# Autodesk Inventor assembly: Printhead Assembly
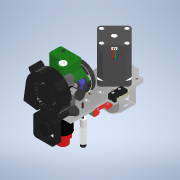
[picture p0: Inventor's stored thumbnail of the model, 180x180]
Saved by Autodesk Inventor 2020 (Build 240168000, 168)
## iProperties
Created: 2023-06-15
Part Number: Printhead Assembly
Document SubType Name: Assembly
Designer: Ishaan
Author: Ishaan
## Documents named in this file (16)
- D:\Documents\Projects\Axiom - IDEX 3D Printer\CAD\01 - Printhead\Printhead Assembly.iam
- D:\Documents\Projects\Axiom - IDEX 3D Printer\CAD\01 - Printhead\Printhead Base Plate REVI.ipt
- D:\Documents\Projects\Axiom - IDEX 3D Printer\CAD\00 - COTS Components\Orbiter Extruder\Orbiter Extruder with Sensor.iam
- D:\Documents\Projects\Axiom - IDEX 3D Printer\CAD\00 - COTS Components\CHC Hotend\TD6S-CHC_mockup.iam
- D:\Documents\Projects\Axiom - IDEX 3D Printer\CAD\00 - COTS Components\3010 Fan\Fan 3010.ipt
- D:\Documents\Projects\Axiom - IDEX 3D Printer\CAD\00 - COTS Components\5015 Fan\Radial-Cooling-Fan-5015-DC12V.iam
- D:\Documents\Projects\Axiom - IDEX 3D Printer\CAD\00 - COTS Components\NEMA 14 - X-Axis Long\14HS20-1504S.ipt
- D:\Documents\Projects\Axiom - IDEX 3D Printer\CAD\00 - COTS Components\MGN12H\MGN12H, LINEAR GUIDE BLOCK.ipt
- D:\Documents\Projects\Axiom - IDEX 3D Printer\CAD\00 - COTS Components\Hardware\624 Bearing.ipt
- D:\Documents\Projects\Axiom - IDEX 3D Printer\CAD\00 - COTS Components\Hardware\1127-8-AL.ipt
- D:\Documents\Projects\Axiom - IDEX 3D Printer\CAD\00 - COTS Components\6mm 20T GT2 Timing Pulley 5mm Bore\6mm 20T GT2 Timing Pulley 5mm Bore.ipt
- D:\Documents\Projects\Axiom - IDEX 3D Printer\CAD\00 - COTS Components\Microswitch\MS085xx02FxxxS1A.ipt
- D:\Documents\Projects\Axiom - IDEX 3D Printer\CAD\00 - COTS Components\PINDA Probe\PINDA_placeholder.ipt
- D:\Documents\Projects\Axiom - IDEX 3D Printer\CAD\01 - Printhead\Idler Shear Brace.ipt
- D:\Documents\Projects\Axiom - IDEX 3D Printer\CAD\00 - COTS Components\Hardware\M4 Shim.ipt
- D:\Documents\Projects\Axiom - IDEX 3D Printer\CAD\01 - Printhead\Front Cowling.ipt
## Components (21 placed, 15 different names)
1. Printhead Base Plate REVI:1 — Insert:1, Insert:2, Insert:3, Mate:1, Mate:2, Mate:4, Insert:4, Insert:5, Insert:6, Insert:7, Insert:15, Insert:18, Mate:7, Insert:19, Insert:20, Insert:21, Insert:22, Insert:27, Insert:28, Angle:1
2. Orbiter Extruder with Sensor:1 [sub-assembly] — Insert:1, Insert:2
3. TD6S-CHC_mockup:1 [sub-assembly] — Insert:3, Mate:1, Mate:2, Mate:3, Flush:1, Flush:2
4. Fan 3010:1 — Mate:3, Mate:4, Flush:1, Mate:9, Flush:3
5. Radial-Cooling-Fan-5015-DC12V:1 [sub-assembly] — Mate:10, Flush:4
6. MGN12H, LINEAR GUIDE BLOCK:1 — Insert:6, Insert:7
7. 14HS20-1504S:1 — Insert:4, Insert:5, Mate:8
8. 624 Bearing:1 — Insert:13, Insert:23
9. 624 Bearing:2 — Insert:13, Insert:17
10. 624 Bearing:3 — Insert:11, Insert:24
11. 624 Bearing:4 — Insert:11, Insert:16
12. 1127-8-AL:1 — Insert:17, Insert:18
13. 1127-8-AL:2 — Insert:15, Insert:16
14. 6mm 20T GT2 Timing Pulley 5mm Bore:1 — Mate:7, Mate:8
15. MS085xx02FxxxS1A:1 — Insert:19, Insert:20
16. MS085xx02FxxxS1A:2 — Insert:21, Insert:22
17. PINDA_placeholder:1 — Flush:2
18. Idler Shear Brace:1 — Insert:25, Insert:26, Insert:27, Insert:28
19. M4 Shim:1 — Insert:24, Insert:25
20. M4 Shim:2 — Insert:23, Insert:26
21. Front Cowling:1 — Mate:9, Flush:3, Angle:1, Mate:10, Flush:4
## Relationships (36: Insert 23, Mate 8, Flush 4, Angle 1)
- Insert:1: Printhead Base Plate REVI:1 ↔ Orbiter Extruder with Sensor:1
- Insert:2: Printhead Base Plate REVI:1 ↔ Orbiter Extruder with Sensor:1
- Insert:3: Printhead Base Plate REVI:1 ↔ TD6S-CHC_mockup:1
- Mate:1: Printhead Base Plate REVI:1 ↔ TD6S-CHC_mockup:1
- Mate:2: Printhead Base Plate REVI:1 ↔ TD6S-CHC_mockup:1
- Mate:3: TD6S-CHC_mockup:1 ↔ Fan 3010:1
- Mate:4 (10 mm): Printhead Base Plate REVI:1 ↔ Fan 3010:1
- Flush:1 (-1 mm): TD6S-CHC_mockup:1 ↔ Fan 3010:1
- Insert:4: Printhead Base Plate REVI:1 ↔ 14HS20-1504S:1
- Insert:5: Printhead Base Plate REVI:1 ↔ 14HS20-1504S:1
- Insert:6: Printhead Base Plate REVI:1 ↔ MGN12H, LINEAR GUIDE BLOCK:1
- Insert:7: Printhead Base Plate REVI:1 ↔ MGN12H, LINEAR GUIDE BLOCK:1
- Insert:11: 624 Bearing:3 ↔ 624 Bearing:4
- Insert:13: 624 Bearing:1 ↔ 624 Bearing:2
- Insert:15: Printhead Base Plate REVI:1 ↔ 1127-8-AL:2
- Insert:16: 624 Bearing:4 ↔ 1127-8-AL:2
- Insert:17: 624 Bearing:2 ↔ 1127-8-AL:1
- Insert:18: Printhead Base Plate REVI:1 ↔ 1127-8-AL:1
- Mate:7: Printhead Base Plate REVI:1 ↔ 6mm 20T GT2 Timing Pulley 5mm Bore:1
- Mate:8: 14HS20-1504S:1 ↔ 6mm 20T GT2 Timing Pulley 5mm Bore:1
- Insert:19: Printhead Base Plate REVI:1 ↔ MS085xx02FxxxS1A:1
- Insert:20: Printhead Base Plate REVI:1 ↔ MS085xx02FxxxS1A:1
- Insert:21: Printhead Base Plate REVI:1 ↔ MS085xx02FxxxS1A:2
- Insert:22: Printhead Base Plate REVI:1 ↔ MS085xx02FxxxS1A:2
- Flush:2 (-1 mm): TD6S-CHC_mockup:1 ↔ PINDA_placeholder:1
- Insert:23: 624 Bearing:1 ↔ M4 Shim:2
- Insert:24: 624 Bearing:3 ↔ M4 Shim:1
- Insert:25: Idler Shear Brace:1 ↔ M4 Shim:1
- Insert:26: Idler Shear Brace:1 ↔ M4 Shim:2
- Insert:27: Printhead Base Plate REVI:1 ↔ Idler Shear Brace:1
- Insert:28: Printhead Base Plate REVI:1 ↔ Idler Shear Brace:1
- Mate:9: Fan 3010:1 ↔ Front Cowling:1
- Flush:3: Fan 3010:1 ↔ Front Cowling:1
- Angle:1 (0 deg): Printhead Base Plate REVI:1 ↔ Front Cowling:1
- Mate:10: Radial-Cooling-Fan-5015-DC12V:1 ↔ Front Cowling:1
- Flush:4: Radial-Cooling-Fan-5015-DC12V:1 ↔ Front Cowling:1
